# Autodesk Inventor assembly: TB_Fullassemb
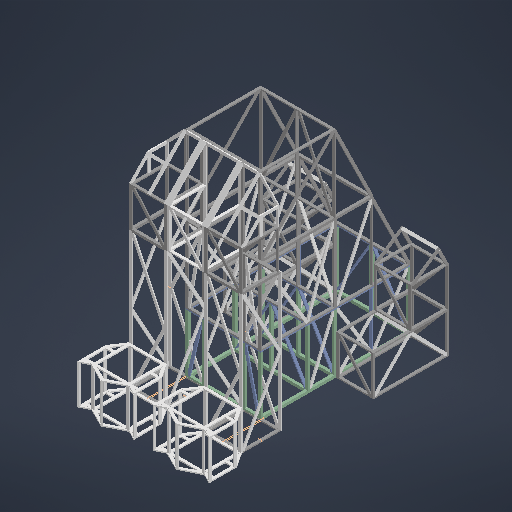
[picture p0: Inventor's stored thumbnail of the model, 512x512]
Saved by Autodesk Inventor 2026 (Build 300175000, 175)
## iProperties
Created: 2025-08-28
Part Number: TB_Fullassemb
Document SubType Name: Assembly
Designer: trott
Author: trott
## Documents named in this file (10)
- C:\Users\trott\Documents\UofSC-ASME-Tiger-Burn-Design-2025\CAD\Assembly\TB_Fullassemb.iam
- C:\Users\trott\Documents\UofSC-ASME-Tiger-Burn-Design-2025\CAD\Body\Base 01\Base 01.iam
- C:\Users\trott\Documents\UofSC-ASME-Tiger-Burn-Design-2025\CAD\Body\Base 02\Base 02.iam
- C:\Users\trott\Documents\UofSC-ASME-Tiger-Burn-Design-2025\CAD\Body\Base 03\Base 03.iam
- C:\Users\trott\Documents\UofSC-ASME-Tiger-Burn-Design-2025\CAD\Legs\Shoulder\Shoulder_L\Shoulder_L.iam
- C:\Users\trott\Documents\UofSC-ASME-Tiger-Burn-Design-2025\CAD\Legs\Shoulder\Shoulder_R\Shoulder_R.iam
- C:\Users\trott\Documents\UofSC-ASME-Tiger-Burn-Design-2025\CAD\Legs\Back Foot\B_Foot.iam
- C:\Users\trott\Documents\UofSC-ASME-Tiger-Burn-Design-2025\CAD\Legs\Back Leg\B_Leg.iam
- C:\Users\trott\Documents\UofSC-ASME-Tiger-Burn-Design-2025\CAD\Legs\Front Leg\F_Leg.iam
- C:\Users\trott\Documents\UofSC-ASME-Tiger-Burn-Design-2025\CAD\Legs\Front Foot\F_Foot.iam
## Components (13 placed, 9 different names)
1. Base 01:1 [sub-assembly] — Mate:1, Flush:1, Flush:2, Flush:8, Mate:5, Flush:9, Mate:6, Flush:10, Flush:11, Flush:12, Mate:8, Flush:13
2. Base 02:1 [sub-assembly] — Mate:1, Flush:1, Flush:2, Mate:2, Flush:3, Flush:4
3. Base 03:1 [sub-assembly] — Mate:2, Flush:3, Flush:4, Flush:5, Flush:6, Mate:3, Mate:4, Flush:7, Mate:10, Flush:14, Mate:11, Mate:12, Mate:13, Mate:14, Flush:15
4. Shoulder_L:1 [sub-assembly] — Flush:5, Flush:6, Mate:3, Mate:10, Flush:14, Mate:11, Mate:15, Flush:16, Flush:17
5. Shoulder_R:1 [sub-assembly] — Mate:4, Flush:7, Mate:12, Mate:13, Mate:14, Flush:15, Mate:16, Flush:18, Flush:19
6. B_Foot:1 [sub-assembly] — Flush:8, Mate:5, Flush:9, Mate:7
7. B_Foot:2 [sub-assembly] — Mate:6, Flush:10, Flush:11, Mate:9
8. B_Leg:1 [sub-assembly] — Mate:7, Flush:12, Mate:8
9. B_Leg:2 [sub-assembly] — Mate:9, Flush:13
10. F_Leg:1 [sub-assembly] — Mate:15, Flush:16, Flush:17, Mate:18, Flush:22, Flush:23
11. F_Leg:2 [sub-assembly] — Mate:16, Flush:18, Flush:19, Mate:17, Flush:20, Flush:21
12. F_Foot:1 [sub-assembly] — Mate:17, Flush:20, Flush:21
13. F_Foot:2 [sub-assembly] — Mate:18, Flush:22, Flush:23
## Relationships (41: Flush 23, Mate 18)
- Mate:1: Base 01:1 ↔ Base 02:1
- Flush:1: Base 01:1 ↔ Base 02:1
- Flush:2: Base 01:1 ↔ Base 02:1
- Mate:2: Base 02:1 ↔ Base 03:1
- Flush:3: Base 02:1 ↔ Base 03:1
- Flush:4: Base 02:1 ↔ Base 03:1
- Flush:5: Base 03:1 ↔ Shoulder_L:1
- Flush:6: Base 03:1 ↔ Shoulder_L:1
- Mate:3: Base 03:1 ↔ Shoulder_L:1
- Mate:4: Base 03:1 ↔ Shoulder_R:1
- Flush:7: Base 03:1 ↔ Shoulder_R:1
- Flush:8: Base 01:1 ↔ B_Foot:1
- Mate:5: Base 01:1 ↔ B_Foot:1
- Flush:9: Base 01:1 ↔ B_Foot:1
- Mate:6: Base 01:1 ↔ B_Foot:2
- Flush:10: Base 01:1 ↔ B_Foot:2
- Flush:11: Base 01:1 ↔ B_Foot:2
- Mate:7: B_Foot:1 ↔ B_Leg:1
- Flush:12: Base 01:1 ↔ B_Leg:1
- Mate:8: Base 01:1 ↔ B_Leg:1
- Mate:9: B_Foot:2 ↔ B_Leg:2
- Flush:13: Base 01:1 ↔ B_Leg:2
- Mate:10: Base 03:1 ↔ Shoulder_L:1
- Flush:14: Base 03:1 ↔ Shoulder_L:1
- Mate:11: Base 03:1 ↔ Shoulder_L:1
- Mate:12: Base 03:1 ↔ Shoulder_R:1
- Mate:13: Base 03:1 ↔ Shoulder_R:1
- Mate:14: Base 03:1 ↔ Shoulder_R:1
- Flush:15: Base 03:1 ↔ Shoulder_R:1
- Mate:15: Shoulder_L:1 ↔ F_Leg:1
- Flush:16: Shoulder_L:1 ↔ F_Leg:1
- Flush:17: Shoulder_L:1 ↔ F_Leg:1
- Mate:16: Shoulder_R:1 ↔ F_Leg:2
- Flush:18: Shoulder_R:1 ↔ F_Leg:2
- Flush:19: Shoulder_R:1 ↔ F_Leg:2
- Mate:17: F_Leg:2 ↔ F_Foot:1
- Flush:20: F_Leg:2 ↔ F_Foot:1
- Flush:21: F_Leg:2 ↔ F_Foot:1
- Mate:18: F_Leg:1 ↔ F_Foot:2
- Flush:22: F_Leg:1 ↔ F_Foot:2
- Flush:23: F_Leg:1 ↔ F_Foot:2
